# Autodesk Inventor assembly: Key
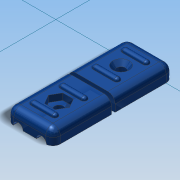
[picture p0: Inventor's stored thumbnail of the model, 180x180]
Saved by Autodesk Inventor 2014 SP2 (Build 180246200, 246)
## iProperties
Created: 2014-06-07
Part Number: Key
Document SubType Name: Assembly
Designer: dliu
Author: dliu
## Documents named in this file (3)
- C:\Users\dliu\Dropbox\dbhome\electric-longboard\dliu\Electronics\Key.iam
- C:\Users\dliu\Dropbox\dbhome\electric-longboard\dliu\Electronics\Solid2_1.ipt
- C:\Users\dliu\Dropbox\dbhome\electric-longboard\dliu\Electronics\Solid3_1.ipt
## Components (2 placed, 2 different names)
1. Solid2_1:1 — Mate:2
2. Solid3_1:1 — Mate:1
## Relationships (2: Mate 2)
- Mate:1: Solid3_1:1
- Mate:2: Solid2_1:1
